# Autodesk Inventor assembly: benchtop-mesoSPIM-V2-1
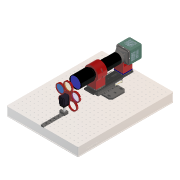
[picture p0: Inventor's stored thumbnail of the model, 180x180]
Saved by Autodesk Inventor 2021 (Build 250183000, 183)
## iProperties
Created: 2020-09-21
Part Number: benchtop-mesoSPIM-V2-1
Document SubType Name: Assembly
Designer: voigt
Author: voigt
## Documents named in this file (68)
- C:\Users\Public\GitHub-public\benchtop-hardware\Benchtop\CAD-model-Inventor2021\mesoSPIM\benchtop-mesoSPIM_latest.iam
- C:\Users\Public\GitHub-public\benchtop-hardware\Benchtop\CAD-model-Inventor2021\library\Thorlabs\breadboards\PBG52522-Step.iam
- C:\Users\Public\GitHub-public\benchtop-hardware\Benchtop\CAD-model-Inventor2021\library\Thorlabs\accessoires\AV6_M.ipt
- C:\Users\Public\GitHub-public\benchtop-hardware\Benchtop\CAD-model-Inventor2021\library\Thorlabs\extrusions\XE25L375_M.ipt
- C:\Users\Public\GitHub-public\benchtop-hardware\Benchtop\CAD-model-Inventor2021\library\Thorlabs\extrusions\RM1S.ipt
- C:\Users\Public\GitHub-public\benchtop-hardware\Benchtop\CAD-model-Inventor2021\library\Thorlabs\extrusions\RM1G.ipt
- C:\Users\Public\GitHub-public\benchtop-hardware\Benchtop\CAD-model-Inventor2021\library\Thorlabs\extrusions\XE25L525_M.ipt
- C:\Users\Public\GitHub-public\benchtop-hardware\Benchtop\CAD-model-Inventor2021\library\Thorlabs\extrusions\XE25L350_M.ipt
- C:\Users\Public\GitHub-public\benchtop-hardware\Benchtop\CAD-model-Inventor2021\library\Thorlabs\accessoires\BBH1.ipt
- C:\Users\Public\GitHub-public\benchtop-hardware\Benchtop\CAD-model-Inventor2021\mesoSPIM\covers\Front_Cover_V1.ipt
- C:\Users\Public\GitHub-public\benchtop-hardware\Benchtop\CAD-model-Inventor2021\library\ASI\LS100_Vertical_Assembly.ipt
- C:\Users\Public\GitHub-public\benchtop-hardware\Benchtop\CAD-model-Inventor2021\library\ASI\LS-50HE ASSEMBLY (Centered Travel).ipt
- C:\Users\Public\GitHub-public\benchtop-hardware\Benchtop\CAD-model-Inventor2021\library\ASI\VTS-2112 DOVE RACK ASSEMBLY - (#DV6010 and #DV6020)_DV6010 ASSEMBLY with CDZ-SLIDE C.iam
- C:\Users\Public\GitHub-public\benchtop-hardware\Benchtop\CAD-model-Inventor2021\library\ASI\LS-50 LE ASSEMBLY_HOME.iam
- C:\Users\Public\GitHub-public\benchtop-hardware\Benchtop\CAD-model-Inventor2021\library\ASI\C60-3060-CMR-1011 - C-MOUNT TO LS50 SLIDE ADAPTER.ipt
- C:\Users\Public\GitHub-public\benchtop-hardware\Benchtop\CAD-model-Inventor2021\library\ASI\C60-3060-CMR - 3060 C-MOUNT ROTATING ASSEMBLY_C60-3060-CMR-Mo-ER20.iam
- C:\Users\Public\GitHub-public\benchtop-hardware\Benchtop\CAD-model-Inventor2021\library\ASI\LS-5012 - LS-BREADBOARD ADAPTER PLATE.ipt
- C:\Users\Public\GitHub-public\benchtop-hardware\Benchtop\CAD-model-Inventor2021\library\Thorlabs\rails\XT66SD.ipt
- C:\Users\Public\GitHub-public\benchtop-hardware\Benchtop\CAD-model-Inventor2021\library\Photometrics\Iris15_Volume_Correct.ipt
- C:\Users\Public\GitHub-public\benchtop-hardware\Benchtop\CAD-model-Inventor2021\library\Thorlabs\rails\XT66P2_M_single.ipt
- C:\Users\Public\GitHub-public\benchtop-hardware\Benchtop\CAD-model-Inventor2021\mesoSPIM\covers\Side_Cover_V1.ipt
- C:\Users\Public\GitHub-public\benchtop-hardware\Benchtop\CAD-model-Inventor2021\mesoSPIM\covers\Top_Cover_V1.ipt
- C:\Users\Public\GitHub-public\benchtop-hardware\Benchtop\CAD-model-Inventor2021\library\Thorlabs\extrusions\XE25H.ipt
- C:\Users\Public\GitHub-public\benchtop-hardware\Benchtop\CAD-model-Inventor2021\library\Thorlabs\30mm_cage_system\cage_plates\CP33_M.ipt
- C:\Users\Public\GitHub-public\benchtop-hardware\Benchtop\CAD-model-Inventor2021\library\Thorlabs\30mm_cage_system\cage_rods\ER8_CageRod.ipt
- C:\Users\Public\GitHub-public\benchtop-hardware\Benchtop\CAD-model-Inventor2021\library\Thorlabs\optics\AC254-060-A-ML.ipt
- C:\Users\Public\GitHub-public\benchtop-hardware\Benchtop\CAD-model-Inventor2021\library\Thorlabs\accessoires\SM1FCA-APC-Fiberadapter.ipt
- C:\Users\Public\GitHub-public\benchtop-hardware\Benchtop\CAD-model-Inventor2021\library\Thorlabs\posts\post_mounts\PH40_M.ipt
- C:\Users\Public\GitHub-public\benchtop-hardware\Benchtop\CAD-model-Inventor2021\library\Thorlabs\posts\12_7_mm_posts\TR40M.ipt
- C:\Users\Public\GitHub-public\benchtop-hardware\Benchtop\CAD-model-Inventor2021\library\Thorlabs\30mm_cage_system\optics_mounts\KCB1E_M.ipt
- C:\Users\Public\GitHub-public\benchtop-hardware\Benchtop\CAD-model-Inventor2021\library\Thorlabs\optics\BBE1-E02-Step.ipt
- C:\Users\Public\GitHub-public\benchtop-hardware\Benchtop\CAD-model-Inventor2021\library\Thorlabs\optics\AC254-100-A-ML.ipt
- C:\Users\Public\GitHub-public\benchtop-hardware\Benchtop\CAD-model-Inventor2021\library\Optotune\EL-16-40\EL-16-40-TC-C (133-193-03-R0-01).iam
- C:\Users\Public\GitHub-public\benchtop-hardware\Benchtop\CAD-model-Inventor2021\library\Thorlabs\30mm_cage_system\SM1_tubes\SM1L10.ipt
- C:\Users\Public\GitHub-public\benchtop-hardware\Benchtop\CAD-model-Inventor2021\library\Thorlabs\accessoires\SM1A9.ipt
- C:\Users\Public\GitHub-public\benchtop-hardware\Benchtop\CAD-model-Inventor2021\library\Thorlabs\accessoires\SM1T2.ipt
- C:\Users\Public\GitHub-public\benchtop-hardware\Benchtop\CAD-model-Inventor2021\library\Thorlabs\accessoires\SM1NT.ipt
- C:\Users\Public\GitHub-public\benchtop-hardware\Benchtop\CAD-model-Inventor2021\library\Thorlabs\stages\XRN-B1_M-Micrometer-Baseplate.ipt
- C:\Users\Public\GitHub-public\benchtop-hardware\Benchtop\CAD-model-Inventor2021\library\Thorlabs\posts\post_mounts\PH75_M-Step.ipt
- C:\Users\Public\GitHub-public\benchtop-hardware\Benchtop\CAD-model-Inventor2021\library\Thorlabs\stages\XLN25P_M.ipt
- C:\Users\Public\GitHub-public\benchtop-hardware\Benchtop\CAD-model-Inventor2021\library\Thorlabs\stages\XRN25P_M.ipt
- C:\Users\Public\GitHub-public\benchtop-hardware\Benchtop\CAD-model-Inventor2021\library\Thorlabs\posts\12_7_mm_posts\TR75M.ipt
- C:\Users\Public\GitHub-public\benchtop-hardware\Benchtop\CAD-model-Inventor2021\mesoSPIM\excitation_path\components\60mm-blank-cageplate-LCP03M-Nikon-MOD.ipt
- C:\Users\Public\GitHub-public\benchtop-hardware\Benchtop\CAD-model-Inventor2021\library\Thorlabs\other\F-Mount-AdapterSM2NFM-Step.ipt
- C:\Users\Public\GitHub-public\benchtop-hardware\Benchtop\CAD-model-Inventor2021\library\Nikon\50mm_1_4G_body_disassembled.ipt
- C:\Users\Public\GitHub-public\benchtop-hardware\Benchtop\CAD-model-Inventor2021\library\Thorlabs\30mm_cage_system\cage_rods\ER4_CageRod.ipt
- C:\Users\Public\GitHub-public\benchtop-hardware\Benchtop\CAD-model-Inventor2021\mesoSPIM\sample_handling\Cuvette-Sampleholder\Cuvette-Sampleholder-with-base.iam
- C:\Users\nvladi\Documents\Inventor\mesoSPIM_design_benchtop_V2\library\Thorlabs\30mm_cage_system\cage_rods\ER_CageRod.ipt
- C:\Users\Public\GitHub-public\benchtop-hardware\Benchtop\CAD-model-Inventor2021\library\Mouse_Brain\mousebrain2.ipt
- C:\Users\Public\GitHub-public\benchtop-hardware\Benchtop\CAD-model-Inventor2021\mesoSPIM\immersion_cuvette_mounts\ImmersionCuvetteAssembly.iam
- C:\Users\Public\GitHub-public\benchtop-hardware\Benchtop\CAD-model-Inventor2021\mesoSPIM\sample_handling\IDISCO-Sampleholder\Clamp-assembly.iam
- C:\Users\Public\GitHub-public\benchtop-hardware\Benchtop\CAD-model-Inventor2021\library\Thorlabs\accessoires\SM1A10.ipt
- C:\Users\Public\GitHub-public\benchtop-hardware\Benchtop\CAD-model-Inventor2021\library\Thorlabs\accessoires\SM1M20.ipt
- C:\Users\Public\GitHub-public\benchtop-hardware\Benchtop\CAD-model-Inventor2021\library\Thorlabs\optics\AC254-060-A-ML_CPY.ipt
- C:\Users\Public\GitHub-public\benchtop-hardware\Benchtop\CAD-model-Inventor2021\library\Thorlabs\accessoires\SM1FCA-APC-Fiberadapter_CPY.ipt
- C:\Users\Public\GitHub-public\benchtop-hardware\Benchtop\CAD-model-Inventor2021\mesoSPIM\detection_path\filter-wheel\FilterWheel-Dynamixel(MX28).iam
- C:\Users\Public\GitHub-public\benchtop-hardware\Benchtop\CAD-model-Inventor2021\library\Thorlabs\rails\RLA150_M.ipt
- C:\Users\Public\GitHub-public\benchtop-hardware\Benchtop\custom-parts\excitation-mirror-bracket\mirror-bracket.ipt
- C:\Users\Public\GitHub-public\benchtop-hardware\Benchtop\CAD-model-Inventor2021\mesoSPIM\excitation_path\15mm-galvo(Thorlabs-QS15)-assembly\15mm-QS15-galvo-assembly.iam
- C:\Users\Public\GitHub-public\benchtop-hardware\Benchtop\CAD-model-Inventor2021\library\ASI\ASI_mesoSPIM_Bridge-wide.ipt
- C:\Users\Public\GitHub-public\benchtop-hardware\Benchtop\CAD-model-Inventor2021\mesoSPIM\detection_path\Mitutoyo\Mitutoyo-BD-Plan-Apo-system.iam
- C:\Users\Public\GitHub-public\benchtop-hardware\Benchtop\custom-parts\detection-objective-mounts\Iris15-XT66P2M.ipt
- C:\Users\Public\GitHub-public\benchtop-hardware\Benchtop\CAD-model-Inventor2021\library\Thorlabs\accessoires\AB90H.ipt
- C:\Users\Public\GitHub-public\benchtop-hardware\Benchtop\custom-parts\detection-objective-mounts\ThorlabsSM2L30-XT66P2M.ipt
- C:\Users\Public\GitHub-public\benchtop-hardware\Benchtop\custom-parts\detection-accessories\Mitutoyo-MT1(tube-lens)-SM2-adapter\AdapterMT1-SM2tube.ipt
- C:\Users\Public\GitHub-public\benchtop-hardware\Benchtop\CAD-model-Inventor2021\library\Thorlabs\kinematic_bases\KB25_M-Step.ipt
- C:\Users\Public\GitHub-public\benchtop-hardware\Benchtop\CAD-model-Inventor2021\library\Lensation\Lensagon-T25M-12-155I.ipt
- C:\Users\Public\GitHub-public\benchtop-hardware\Benchtop\CAD-model-Inventor2021\mesoSPIM\detection_path\filter-wheel\Filter.ipt
## Components (146 placed, 66 different names)
1. Filter:1 — Flush:83
2. Filter:2 — Insert:27
3. Filter:3 — Insert:26
4. AV6_M:4 — Mate:6, Mate:7
5. AV6_M:3 — Mate:8, Mate:9
6. AV6_M:2 — Mate:12, Mate:13
7. AV6_M:1 — Mate:10, Mate:11
8. PBG52522-Step:1 [sub-assembly] — Flush:1, Flush:2, Mate:5, Mate:6, Mate:7, Mate:8, Mate:9, Mate:10, Mate:11, Mate:12, Mate:13, Mate:14, Mate:15, Angle:1, Mate:16, Mate:17, Angle:2, Mate:18, Mate:19, Angle:3, Mate:20, Mate:21, Angle:4, Mate:32, Mate:48, Mate:49, Angle:5, Angle:6, Mate:72, Flush:45, Mate:139, Mate:140, Angle:18, Mate:141, Mate:142, Angle:19, Flush:49, Angle:20, Mate:191, Mate:192, Angle:23, Angle:24, Mate:196, Mate:197, Mate:198, Angle:25, Mate:199, Mate:200, Angle:26, Mate:238, Mate:239, Angle:28, Angle:30, Mate:243, Angle:44, Mate:385, Angle:47, Insert:19, Angle:48, Angle:49, Angle:50, Flush:74, Flush:75, Mate:392, Mate:395, Mate:397, Mate:398
9. TR40M:5 — Mate:367, VerticalPos, Insert:9
10. LS100_Vertical_Assembly:1 — Mate:48, Angle:5, Mate:52, Flush:74, Mate:391, Mate:393, Mate:394, Flush:78
11. LS100_Vertical_Assembly:2 — Mate:49, Angle:6, Flush:75, Mate:396, Flush:79, Mate:399, Flush:80
12. ASI_mesoSPIM_Bridge-wide:1 — Mate:52, Mate:55, Flush:36
13. LS-50HE ASSEMBLY (Centered Travel):1 — Mate:55, Flush:36, Mate:56, Mate:57, Angle:7, Mate:58, Mate:59, Angle:8
14. AB90H:1 — Mate:394, Mate:395, Flush:78
15. AB90H:2 — Mate:391, Mate:392, Mate:393
16. AB90H:3 — Mate:396, Flush:79, Mate:397
17. AB90H:4 — Mate:398, Mate:399, Flush:80
18. VTS-2112 DOVE RACK ASSEMBLY - (#DV6010 and #DV6020)_DV6010 ASSEMBLY with CDZ-SLIDE C:1 [sub-assembly] — Mate:57, Angle:7, Mate:58, Mate:59, Mate:60, Mate:61, Mate:62
19. LS-50 LE ASSEMBLY_HOME:1 [sub-assembly] — Mate:60, Mate:61, Mate:62, Angle:8, Mate:63, Mate:64, Mate:65
20. C60-3060-CMR-1011 - C-MOUNT TO LS50 SLIDE ADAPTER:1 — Mate:63, Mate:64, Mate:65, Mate:66, Mate:67
21. C60-3060-CMR - 3060 C-MOUNT ROTATING ASSEMBLY_C60-3060-CMR-Mo-ER20:1 [sub-assembly] — Mate:66, Mate:67, Mate:367, VerticalPos
22. AdapterMT1-SM2tube:1
23. ThorlabsSM2L30-XT66P2M:1 — Mate:400, Flush:81, Flush:82
24. Lensagon-T25M-12-155I:1 — Insert:25
25. Mitutoyo-BD-Plan-Apo-system:1 [sub-assembly] — Insert:24
26. Iris15-XT66P2M:1 — Mate:390, Flush:76, Flush:77
27. Iris15_Volume_Correct:1 — Angle:11, Insert:24, Insert:25
28. XT66P2_M_single:1 — Mate:82, Mate:83, Mate:390, Flush:76, Flush:77
29. XT66P2_M_single:2 — Mate:84, Mate:85, Mate:400, Flush:81, Flush:82
30. 15mm-QS15-galvo-assembly:1 [sub-assembly] — Insert:21
31. mirror-bracket:1 — Mate:389, Angle:50
32. SM1M20:1 — Insert:15, Insert:17
33. SM1A10:1 — Insert:12, Insert:14
34. SM1FCA-APC-Fiberadapter:1 — Insert:17
35. AC254-060-A-ML:1 — Insert:14, Insert:15
36. 60mm-blank-cageplate-LCP03M-Nikon-MOD:1 — Mate:344, Mate:345, Mate:347, Flush:66, Mate:350, Flush:67, Insert:1
37. F-Mount-AdapterSM2NFM-Step:1 — Mate:344, Mate:345, Mate:346
38. 50mm_1_4G_body_disassembled:1 — Mate:346, Mate:347
39. TR75M:2 — Mate:272
40. KCB1E_M:4 — Mate:254, Mate:255, Mate:258, Mate:259, Mate:389
41. BBE1-E02-Step:5 — Mate:258, Mate:259
42. XRN25P_M:2
43. PH75_M-Step:2 — Mate:192, Angle:23, Mate:272
44. XRN-B1_M-Micrometer-Baseplate:1 — Mate:191, Angle:24, Mate:196
45. EL-16-40-TC-C (133-193-03-R0-01):1 [sub-assembly] — Mate:175, Mate:178, Mate:179, Insert:12
46. SM1L10:2 — Mate:177, Mate:181, Mate:182, Mate:183
47. SM1A9:1 — Mate:178, Mate:179, Mate:180
48. SM1T2:1 — Mate:180, Mate:181
49. SM1NT:1 — Mate:182, Mate:183
50. PH40_M:1 — Mate:139, Mate:140, Angle:18, Mate:148
51. PH40_M:2 — Mate:141, Mate:142, Angle:19, Mate:150
52. CP33_M:5 — Mate:147, Mate:148, Mate:153, Mate:154, Mate:155, Mate:156, Flush:53, Mate:159, Mate:160, Angle:51
53. CP33_M:6 — Mate:149, Mate:150, Mate:161, Mate:162
54. CP33_M:13 — Insert:22, Insert:23, Angle:51
55. CP33_M:7 — Mate:151, Mate:157, Flush:54, Mate:169
56. ER8_CageRod:4 — Mate:156, Flush:51
57. ER8_CageRod:5 — Mate:155, Flush:50, Flush:51, Flush:52, Mate:157, Insert:23
58. ER8_CageRod:6 — Mate:154, Flush:52
59. ER8_CageRod:7 — Mate:153, Flush:50, Flush:53, Flush:54, Mate:164, Mate:165
60. TR40M:1 — Mate:159, Mate:160
61. TR40M:2 — Mate:161, Mate:162
62. KCB1E_M:1 — Mate:163, Mate:164, Mate:165, Mate:167, Mate:175, Mate:177
63. BBE1-E02-Step:1 — Mate:166, Mate:167, Angle:20
64. AC254-100-A-ML:1 — Mate:168, Mate:169
65. AC254-100-A-ML:2 — Insert:22
66. ER4_CageRod:12 — Flush:66
67. ER4_CageRod:19 — Insert:1
68. ER4_CageRod:20
69. ER4_CageRod:13 — Mate:350, Flush:67, Insert:21
70. 15mm-QS15-galvo-assembly:2 [sub-assembly] — Insert:20
71. mirror-bracket:2 — Mate:388, Angle:49
72. SM1FCA-APC-Fiberadapter_CPY:1 — Insert:18
73. AC254-060-A-ML_CPY:1 — Insert:16
74. SM1M20:2 — Insert:16, Insert:18
75. SM1A10:2 — Insert:13
76. 60mm-blank-cageplate-LCP03M-Nikon-MOD:2 — Mate:358, Mate:359, Mate:361, Mate:365, Flush:70, Flush:71, Mate:366
77. F-Mount-AdapterSM2NFM-Step:2 — Mate:358, Mate:359, Mate:360
78. 50mm_1_4G_body_disassembled:2 — Mate:360, Mate:361
79. ER4_CageRod:14 — Mate:365, Flush:70
80. ER4_CageRod:16 — Flush:71, Mate:366, Insert:20
81. TR75M:4 — Mate:278
82. KCB1E_M:5 — Mate:256, Mate:261, Mate:388
83. BBE1-E02-Step:4 — Mate:261
84. XLN25P_M:1 — Mate:403
85. PH40_M:3 — Mate:197, Mate:198, Angle:25, Mate:205
86. PH40_M:4 — Mate:199, Mate:200, Angle:26, Mate:206
87. CP33_M:9 — Mate:201, Mate:205, Mate:207, Mate:208, Mate:211, Mate:212, Mate:213, Mate:214
88. CP33_M:10 — Mate:202, Mate:206, Mate:209, Mate:210, Flush:58
89. TR40M:3 — Mate:207, Mate:208
90. TR40M:4 — Mate:209, Mate:210
91. ER8_CageRod:8 — Mate:211, Flush:57, Flush:59
92. ER8_CageRod:9 — Mate:213, Flush:56, Flush:58, Mate:216, Mate:217, Mate:222
93. ER8_CageRod:10 — Mate:214, Flush:55, Flush:56, Flush:57
94. ER8_CageRod:11 — Mate:212, Flush:55
95. ER4_CageRod:21
96. ER4_CageRod:22
97. KCB1E_M:3 — Mate:215, Mate:216, Mate:217, Mate:219, Angle:27, Mate:227, Mate:228, Mate:229, Mate:231
98. BBE1-E02-Step:3 — Mate:218, Mate:219, Angle:27
99. CP33_M:11 — Mate:220, Flush:59, Mate:224
100. CP33_M:12 — Mate:221, Mate:222, Mate:226
101. AC254-100-A-ML:3 — Mate:223, Mate:224
102. AC254-100-A-ML:4 — Mate:225, Mate:226, Mate:227
103. SM1L10:3 — Mate:228, Mate:229, Mate:230, Mate:236, Mate:237
104. EL-16-40-TC-C (133-193-03-R0-01):2 [sub-assembly] — Mate:230, Mate:231, Mate:232, Mate:233, Insert:13
105. SM1A9:3 — Mate:232, Mate:233, Mate:234, Mate:235
106. SM1T2:2 — Mate:234, Mate:235
107. SM1NT:2 — Mate:236, Mate:237
108. XRN-B1_M-Micrometer-Baseplate:2 — Mate:238, Angle:30, Mate:243, Mate:403
109. PH75_M-Step:3 — Mate:239, Angle:28, Mate:278
110. mousebrain2:1
111. ImmersionCuvetteAssembly:1 [sub-assembly] — Mate:385
112. Clamp-assembly:1 [sub-assembly] — Insert:9, Angle:47
113. KB25_M-Step:1
114. Cuvette-Sampleholder-with-base:1 [sub-assembly] — Angle:44
115. RLA150_M:1 — Insert:19, Angle:48, Mate:386, Mate:387
116. FilterWheel-Dynamixel(MX28):1 [sub-assembly] — Mate:386, Mate:387, Flush:83, Insert:26, Insert:27
117. XE25H:1 — Mate:103, Angle:14, Mate:104, Flush:43
118. XE25H:2 — Mate:105, Mate:106, Flush:44
119. XE25L525_M:1 — Mate:29, Flush:17, Flush:18, Mate:101, Flush:40, Flush:42
120. XE25L525_M:2 — Mate:28, Flush:15, Flush:16, Mate:100, Flush:38
121. XE25L375_M:5 — Mate:27, Flush:13, Flush:14, Flush:19, Mate:30, Flush:20, Mate:103, Flush:43, Mate:105, Flush:44
122. XE25L375_M:6 — Mate:26, Flush:11, Flush:12, Flush:41
123. RM1G:1 — Mate:22, Flush:3, Flush:4, Mate:28, Flush:15, Flush:16
124. RM1G:2 — Mate:24, Flush:7, Flush:8, Mate:26, Flush:11, Flush:12, Mate:29, Flush:17, Flush:18
125. RM1G:3 — Mate:25, Flush:9, Flush:10, Mate:27, Flush:13, Flush:14, Mate:104
126. RM1G:4 — Mate:23, Flush:5, Flush:6, Mate:102, Mate:106
127. XE25L375_M:1 — Mate:14, Mate:15, Angle:1, Mate:22, Flush:3, Flush:4, Flush:37
128. XE25L375_M:2 — Mate:16, Mate:17, Angle:2, Mate:24, Flush:7, Flush:8, Flush:39
129. XE25L375_M:3 — Mate:18, Mate:19, Angle:3, Mate:25, Flush:9, Flush:10
130. XE25L375_M:4 — Mate:20, Mate:21, Angle:4, Mate:23, Flush:5, Flush:6, Flush:21, Mate:31
131. Front_Cover_V1:1 — Mate:41, Mate:42, Mate:43
132. BBH1:1 — Mate:39, Flush:35, Mate:40
133. RM1S:1 — Mate:33, Flush:22, Flush:23
134. RM1S:2 — Mate:34, Flush:24, Flush:25, Flush:33, Flush:34, Mate:38
135. RM1S:3 — Flush:28, Mate:36, Flush:29, Flush:30, Mate:37, Flush:31, Flush:32
136. RM1S:4 — Mate:35, Flush:26, Flush:27
137. XE25L375_M:7 — Flush:19, Mate:30, Flush:20, Mate:34, Flush:24, Flush:25, Flush:28, Mate:36, Flush:29, Flush:30, Mate:43, Angle:14
138. XE25L375_M:8 — Flush:21, Mate:31, Mate:32, Mate:33, Flush:22, Flush:23, Mate:35, Flush:26, Flush:27, Mate:39, Flush:35
139. XE25L350_M:1 — Mate:37, Flush:31, Flush:32, Mate:41, Mate:42
140. XE25L350_M:2 — Flush:33, Flush:34, Mate:38
141. Side_Cover_V1:1 — Mate:100, Flush:37, Flush:38
142. Side_Cover_V1:2 — Mate:101, Flush:39, Flush:40
143. Top_Cover_V1:1 — Mate:102, Flush:41, Flush:42
144. LS-5012 - LS-BREADBOARD ADAPTER PLATE:1 — Mate:70, Angle:9, Mate:72, Mate:77
145. LS-50 LE ASSEMBLY_HOME:2 [sub-assembly] — Mate:70, Angle:9, Mate:73, Mate:74, Angle:10, Mate:77
146. XT66SD:1 — Mate:73, Mate:74, Angle:10, Mate:75, Mate:76, Angle:11, Mate:82, Mate:83, Mate:84, Mate:85
## Relationships (325: Mate 206, Flush 72, Angle 29, Insert 18)
- Flush:1 (135 mm): PBG52522-Step:1
- Flush:2 (225 mm): PBG52522-Step:1
- Mate:5 (-100 mm): PBG52522-Step:1
- Mate:6: AV6_M:4 ↔ PBG52522-Step:1
- Mate:7: AV6_M:4 ↔ PBG52522-Step:1
- Mate:8: AV6_M:3 ↔ PBG52522-Step:1
- Mate:9: AV6_M:3 ↔ PBG52522-Step:1
- Mate:10: AV6_M:1 ↔ PBG52522-Step:1
- Mate:11: AV6_M:1 ↔ PBG52522-Step:1
- Mate:12: AV6_M:2 ↔ PBG52522-Step:1
- Mate:13: AV6_M:2 ↔ PBG52522-Step:1
- Mate:14: PBG52522-Step:1 ↔ XE25L375_M:1
- Mate:15: PBG52522-Step:1 ↔ XE25L375_M:1
- Angle:1 (0 deg): PBG52522-Step:1 ↔ XE25L375_M:1
- Mate:16: PBG52522-Step:1 ↔ XE25L375_M:2
- Mate:17: PBG52522-Step:1 ↔ XE25L375_M:2
- Angle:2 (0 deg): PBG52522-Step:1 ↔ XE25L375_M:2
- Mate:18: PBG52522-Step:1 ↔ XE25L375_M:3
- Mate:19: PBG52522-Step:1 ↔ XE25L375_M:3
- Angle:3 (0 deg): PBG52522-Step:1 ↔ XE25L375_M:3
- Mate:20: PBG52522-Step:1 ↔ XE25L375_M:4
- Mate:21: PBG52522-Step:1 ↔ XE25L375_M:4
- Angle:4 (0 deg): PBG52522-Step:1 ↔ XE25L375_M:4
- Mate:22: RM1G:1 ↔ XE25L375_M:1
- Flush:3: RM1G:1 ↔ XE25L375_M:1
- Flush:4: RM1G:1 ↔ XE25L375_M:1
- Mate:23: RM1G:4 ↔ XE25L375_M:4
- Flush:5: RM1G:4 ↔ XE25L375_M:4
- Flush:6: RM1G:4 ↔ XE25L375_M:4
- Mate:24: RM1G:2 ↔ XE25L375_M:2
- Flush:7: RM1G:2 ↔ XE25L375_M:2
- Flush:8: RM1G:2 ↔ XE25L375_M:2
- Mate:25: RM1G:3 ↔ XE25L375_M:3
- Flush:9: RM1G:3 ↔ XE25L375_M:3
- Flush:10: RM1G:3 ↔ XE25L375_M:3
- Mate:26: XE25L375_M:6 ↔ RM1G:2
- Flush:11: XE25L375_M:6 ↔ RM1G:2
- Flush:12: XE25L375_M:6 ↔ RM1G:2
- Mate:27: XE25L375_M:5 ↔ RM1G:3
- Flush:13: XE25L375_M:5 ↔ RM1G:3
- Flush:14: XE25L375_M:5 ↔ RM1G:3
- Mate:28: XE25L525_M:2 ↔ RM1G:1
- Flush:15: XE25L525_M:2 ↔ RM1G:1
- Flush:16: XE25L525_M:2 ↔ RM1G:1
- Mate:29: XE25L525_M:1 ↔ RM1G:2
- Flush:17: XE25L525_M:1 ↔ RM1G:2
- Flush:18: XE25L525_M:1 ↔ RM1G:2
- Flush:19: XE25L375_M:5 ↔ XE25L375_M:7
- Mate:30: XE25L375_M:5 ↔ XE25L375_M:7
- Flush:20: XE25L375_M:5 ↔ XE25L375_M:7
- Flush:21 (-25 mm): XE25L375_M:4 ↔ XE25L375_M:8
- Mate:31: XE25L375_M:4 ↔ XE25L375_M:8
- Mate:32: PBG52522-Step:1 ↔ XE25L375_M:8
- Mate:33: RM1S:1 ↔ XE25L375_M:8
- Flush:22: RM1S:1 ↔ XE25L375_M:8
- Flush:23: RM1S:1 ↔ XE25L375_M:8
- Mate:34: RM1S:2 ↔ XE25L375_M:7
- Flush:24: RM1S:2 ↔ XE25L375_M:7
- Flush:25: RM1S:2 ↔ XE25L375_M:7
- Mate:35: RM1S:4 ↔ XE25L375_M:8
- Flush:26: RM1S:4 ↔ XE25L375_M:8
- Flush:27: RM1S:4 ↔ XE25L375_M:8
- Flush:28: RM1S:3 ↔ XE25L375_M:7
- Mate:36: RM1S:3 ↔ XE25L375_M:7
- Flush:29: RM1S:3 ↔ XE25L375_M:7
- Flush:30: RM1S:3 ↔ XE25L375_M:7
- Mate:37: RM1S:3 ↔ XE25L350_M:1
- Flush:31: RM1S:3 ↔ XE25L350_M:1
- Flush:32: RM1S:3 ↔ XE25L350_M:1
- Flush:33: RM1S:2 ↔ XE25L350_M:2
- Flush:34: RM1S:2 ↔ XE25L350_M:2
- Mate:38: RM1S:2 ↔ XE25L350_M:2
- Mate:39: BBH1:1 ↔ XE25L375_M:8
- Flush:35: BBH1:1 ↔ XE25L375_M:8
- Mate:40 (62.5 mm): BBH1:1
- Mate:41: Front_Cover_V1:1 ↔ XE25L350_M:1
- Mate:42 (-6 mm): Front_Cover_V1:1 ↔ XE25L350_M:1
- Mate:43 (-2 mm): Front_Cover_V1:1 ↔ XE25L375_M:7
- Mate:44
- Mate:45
- Mate:48: PBG52522-Step:1 ↔ LS100_Vertical_Assembly:1
- Mate:49: PBG52522-Step:1 ↔ LS100_Vertical_Assembly:2
- Angle:5 (0 deg): PBG52522-Step:1 ↔ LS100_Vertical_Assembly:1
- Angle:6 (0 deg): PBG52522-Step:1 ↔ LS100_Vertical_Assembly:2
- Mate:52: LS100_Vertical_Assembly:1 ↔ ASI_mesoSPIM_Bridge-wide:1
- Mate:55: ASI_mesoSPIM_Bridge-wide:1 ↔ LS-50HE ASSEMBLY (Centered Travel):1
- Flush:36: ASI_mesoSPIM_Bridge-wide:1 ↔ LS-50HE ASSEMBLY (Centered Travel):1
- Mate:56 (12.5 mm): LS-50HE ASSEMBLY (Centered Travel):1
- Mate:57: LS-50HE ASSEMBLY (Centered Travel):1 ↔ VTS-2112 DOVE RACK ASSEMBLY - (#DV6010 and #DV6020)_DV6010 ASSEMBLY with CDZ-SLIDE C:1
- Angle:7 (0 deg): LS-50HE ASSEMBLY (Centered Travel):1 ↔ VTS-2112 DOVE RACK ASSEMBLY - (#DV6010 and #DV6020)_DV6010 ASSEMBLY with CDZ-SLIDE C:1
- Mate:58: LS-50HE ASSEMBLY (Centered Travel):1 ↔ VTS-2112 DOVE RACK ASSEMBLY - (#DV6010 and #DV6020)_DV6010 ASSEMBLY with CDZ-SLIDE C:1
- Mate:59: LS-50HE ASSEMBLY (Centered Travel):1 ↔ VTS-2112 DOVE RACK ASSEMBLY - (#DV6010 and #DV6020)_DV6010 ASSEMBLY with CDZ-SLIDE C:1
- Mate:60: VTS-2112 DOVE RACK ASSEMBLY - (#DV6010 and #DV6020)_DV6010 ASSEMBLY with CDZ-SLIDE C:1 ↔ LS-50 LE ASSEMBLY_HOME:1
- Mate:61: VTS-2112 DOVE RACK ASSEMBLY - (#DV6010 and #DV6020)_DV6010 ASSEMBLY with CDZ-SLIDE C:1 ↔ LS-50 LE ASSEMBLY_HOME:1
- Mate:62: VTS-2112 DOVE RACK ASSEMBLY - (#DV6010 and #DV6020)_DV6010 ASSEMBLY with CDZ-SLIDE C:1 ↔ LS-50 LE ASSEMBLY_HOME:1
- Angle:8 (0 deg): LS-50HE ASSEMBLY (Centered Travel):1 ↔ LS-50 LE ASSEMBLY_HOME:1
- Mate:63: LS-50 LE ASSEMBLY_HOME:1 ↔ C60-3060-CMR-1011 - C-MOUNT TO LS50 SLIDE ADAPTER:1
- Mate:64: LS-50 LE ASSEMBLY_HOME:1 ↔ C60-3060-CMR-1011 - C-MOUNT TO LS50 SLIDE ADAPTER:1
- Mate:65: LS-50 LE ASSEMBLY_HOME:1 ↔ C60-3060-CMR-1011 - C-MOUNT TO LS50 SLIDE ADAPTER:1
- Mate:66: C60-3060-CMR-1011 - C-MOUNT TO LS50 SLIDE ADAPTER:1 ↔ C60-3060-CMR - 3060 C-MOUNT ROTATING ASSEMBLY_C60-3060-CMR-Mo-ER20:1
- Mate:67: C60-3060-CMR-1011 - C-MOUNT TO LS50 SLIDE ADAPTER:1 ↔ C60-3060-CMR - 3060 C-MOUNT ROTATING ASSEMBLY_C60-3060-CMR-Mo-ER20:1
- Mate:70: LS-5012 - LS-BREADBOARD ADAPTER PLATE:1 ↔ LS-50 LE ASSEMBLY_HOME:2
- Angle:9 (0 deg): LS-5012 - LS-BREADBOARD ADAPTER PLATE:1 ↔ LS-50 LE ASSEMBLY_HOME:2
- Mate:72: PBG52522-Step:1 ↔ LS-5012 - LS-BREADBOARD ADAPTER PLATE:1
- Mate:73: LS-50 LE ASSEMBLY_HOME:2 ↔ XT66SD:1
- Mate:74: LS-50 LE ASSEMBLY_HOME:2 ↔ XT66SD:1
- Angle:10 (0 deg): LS-50 LE ASSEMBLY_HOME:2 ↔ XT66SD:1
- Mate:75: XT66SD:1
- Mate:76: XT66SD:1
- Mate:77: LS-5012 - LS-BREADBOARD ADAPTER PLATE:1 ↔ LS-50 LE ASSEMBLY_HOME:2
- Angle:11 (0 deg): Iris15_Volume_Correct:1 ↔ XT66SD:1
- Mate:82: XT66P2_M_single:1 ↔ XT66SD:1
- Mate:83: XT66P2_M_single:1 ↔ XT66SD:1
- Mate:84: XT66P2_M_single:2 ↔ XT66SD:1
- Mate:85: XT66P2_M_single:2 ↔ XT66SD:1
- Mate:100: XE25L525_M:2 ↔ Side_Cover_V1:1
- Flush:37: XE25L375_M:1 ↔ Side_Cover_V1:1
- Flush:38: XE25L525_M:2 ↔ Side_Cover_V1:1
- Mate:101: XE25L525_M:1 ↔ Side_Cover_V1:2
- Flush:39: XE25L375_M:2 ↔ Side_Cover_V1:2
- Flush:40: XE25L525_M:1 ↔ Side_Cover_V1:2
- Mate:102: RM1G:4 ↔ Top_Cover_V1:1
- Flush:41: XE25L375_M:6 ↔ Top_Cover_V1:1
- Flush:42: XE25L525_M:1 ↔ Top_Cover_V1:1
- Mate:103: XE25H:1 ↔ XE25L375_M:5
- Angle:14 (0 deg): XE25H:1 ↔ XE25L375_M:7
- Mate:104: XE25H:1 ↔ RM1G:3
- Flush:43 (5.75 mm): XE25H:1 ↔ XE25L375_M:5
- Mate:105: XE25H:2 ↔ XE25L375_M:5
- Mate:106: XE25H:2 ↔ RM1G:4
- Flush:44 (5.75 mm): XE25H:2 ↔ XE25L375_M:5
- Flush:45 (215 mm): PBG52522-Step:1
- Flush:46 (-100 mm)
- Flush:47 (100 mm)
- Mate:139: PBG52522-Step:1 ↔ PH40_M:1
- Mate:140: PBG52522-Step:1 ↔ PH40_M:1
- Angle:18 (0 deg): PBG52522-Step:1 ↔ PH40_M:1
- Mate:141: PBG52522-Step:1 ↔ PH40_M:2
- Mate:142: PBG52522-Step:1 ↔ PH40_M:2
- Angle:19 (0 deg): PBG52522-Step:1 ↔ PH40_M:2
- Flush:49 (70 mm): PBG52522-Step:1
- Mate:143
- Mate:144
- Mate:145
- Mate:146
- Mate:147: CP33_M:5
- Mate:148: PH40_M:1 ↔ CP33_M:5
- Mate:149: CP33_M:6
- Mate:150: PH40_M:2 ↔ CP33_M:6
- Mate:151: CP33_M:7
- Mate:153: CP33_M:5 ↔ ER8_CageRod:7
- Mate:154: CP33_M:5 ↔ ER8_CageRod:6
- Mate:155: CP33_M:5 ↔ ER8_CageRod:5
- Mate:156: CP33_M:5 ↔ ER8_CageRod:4
- Flush:50: ER8_CageRod:5 ↔ ER8_CageRod:7
- Flush:51: ER8_CageRod:4 ↔ ER8_CageRod:5
- Flush:52: ER8_CageRod:5 ↔ ER8_CageRod:6
- Flush:53 (-39 mm): CP33_M:5 ↔ ER8_CageRod:7
- Mate:157: CP33_M:7 ↔ ER8_CageRod:5
- Mate:159: CP33_M:5 ↔ TR40M:1
- Mate:160: CP33_M:5 ↔ TR40M:1
- Mate:161: CP33_M:6 ↔ TR40M:2
- Mate:162: CP33_M:6 ↔ TR40M:2
- Flush:54: CP33_M:7 ↔ ER8_CageRod:7
- Mate:163: KCB1E_M:1
- Mate:164: ER8_CageRod:7 ↔ KCB1E_M:1
- Mate:165: ER8_CageRod:7 ↔ KCB1E_M:1
- Mate:166: BBE1-E02-Step:1
- Mate:167: KCB1E_M:1 ↔ BBE1-E02-Step:1
- Angle:20 (-90 deg): PBG52522-Step:1 ↔ BBE1-E02-Step:1
- Mate:168: AC254-100-A-ML:1
- Mate:169: CP33_M:7 ↔ AC254-100-A-ML:1
- Mate:175 (35.6 mm): EL-16-40-TC-C (133-193-03-R0-01):1 ↔ KCB1E_M:1
- Mate:177: SM1L10:2 ↔ KCB1E_M:1
- Mate:178: EL-16-40-TC-C (133-193-03-R0-01):1 ↔ SM1A9:1
- Mate:179: EL-16-40-TC-C (133-193-03-R0-01):1 ↔ SM1A9:1
- Mate:180: SM1A9:1 ↔ SM1T2:1
- Mate:181: SM1L10:2 ↔ SM1T2:1
- Mate:182: SM1L10:2 ↔ SM1NT:1
- Mate:183: SM1L10:2 ↔ SM1NT:1
- Mate:191: PBG52522-Step:1 ↔ XRN-B1_M-Micrometer-Baseplate:1
- Mate:192: PBG52522-Step:1 ↔ PH75_M-Step:2
- Angle:23 (0 deg): PBG52522-Step:1 ↔ PH75_M-Step:2
- Angle:24 (0 deg): PBG52522-Step:1 ↔ XRN-B1_M-Micrometer-Baseplate:1
- Mate:196: PBG52522-Step:1 ↔ XRN-B1_M-Micrometer-Baseplate:1
- Mate:197: PBG52522-Step:1 ↔ PH40_M:3
- Mate:198: PBG52522-Step:1 ↔ PH40_M:3
- Angle:25 (0 deg): PBG52522-Step:1 ↔ PH40_M:3
- Mate:199: PBG52522-Step:1 ↔ PH40_M:4
- Mate:200: PBG52522-Step:1 ↔ PH40_M:4
- Angle:26 (0 deg): PBG52522-Step:1 ↔ PH40_M:4
- Mate:201: CP33_M:9
- Mate:202: CP33_M:10
- Mate:205: PH40_M:3 ↔ CP33_M:9
- Mate:206: PH40_M:4 ↔ CP33_M:10
- Mate:207: CP33_M:9 ↔ TR40M:3
- Mate:208: CP33_M:9 ↔ TR40M:3
- Mate:209: CP33_M:10 ↔ TR40M:4
- Mate:210: CP33_M:10 ↔ TR40M:4
- Mate:211: CP33_M:9 ↔ ER8_CageRod:8
- Mate:212: CP33_M:9 ↔ ER8_CageRod:11
- Mate:213: CP33_M:9 ↔ ER8_CageRod:9
- Mate:214: CP33_M:9 ↔ ER8_CageRod:10
- Flush:55: ER8_CageRod:10 ↔ ER8_CageRod:11
- Flush:56: ER8_CageRod:9 ↔ ER8_CageRod:10
- Flush:57: ER8_CageRod:8 ↔ ER8_CageRod:10
- Flush:58 (-39 mm): CP33_M:10 ↔ ER8_CageRod:9
- Mate:215: KCB1E_M:3
- Mate:216: ER8_CageRod:9 ↔ KCB1E_M:3
- Mate:217: ER8_CageRod:9 ↔ KCB1E_M:3
- Mate:218: BBE1-E02-Step:3
- Mate:219: KCB1E_M:3 ↔ BBE1-E02-Step:3
- Angle:27 (0 deg): KCB1E_M:3 ↔ BBE1-E02-Step:3
- Mate:220: CP33_M:11
- Mate:221: CP33_M:12
- Mate:222: ER8_CageRod:9 ↔ CP33_M:12
- Flush:59: ER8_CageRod:8 ↔ CP33_M:11
- Mate:223: AC254-100-A-ML:3
- Mate:224: CP33_M:11 ↔ AC254-100-A-ML:3
- Mate:225: AC254-100-A-ML:4
- Mate:226: CP33_M:12 ↔ AC254-100-A-ML:4
- Mate:227 (0.5 mm): KCB1E_M:3 ↔ AC254-100-A-ML:4
- Mate:228: KCB1E_M:3 ↔ SM1L10:3
- Mate:229: KCB1E_M:3 ↔ SM1L10:3
- Mate:230: SM1L10:3 ↔ EL-16-40-TC-C (133-193-03-R0-01):2
- Mate:231 (35.6 mm): KCB1E_M:3 ↔ EL-16-40-TC-C (133-193-03-R0-01):2
- Mate:232: EL-16-40-TC-C (133-193-03-R0-01):2 ↔ SM1A9:3
- Mate:233: EL-16-40-TC-C (133-193-03-R0-01):2 ↔ SM1A9:3
- Mate:234: SM1A9:3 ↔ SM1T2:2
- Mate:235: SM1A9:3 ↔ SM1T2:2
- Mate:236: SM1L10:3 ↔ SM1NT:2
- Mate:237: SM1L10:3 ↔ SM1NT:2
- Mate:238: PBG52522-Step:1 ↔ XRN-B1_M-Micrometer-Baseplate:2
- Mate:239: PBG52522-Step:1 ↔ PH75_M-Step:3
- Angle:28 (0 deg): PBG52522-Step:1 ↔ PH75_M-Step:3
- Angle:30 (0 deg): PBG52522-Step:1 ↔ XRN-B1_M-Micrometer-Baseplate:2
- Mate:243: PBG52522-Step:1 ↔ XRN-B1_M-Micrometer-Baseplate:2
- [Mate]: XRN25P_M:2 ↔ XRN-B1_M-Micrometer-Baseplate:1
- [Mate]: XRN25P_M:2 ↔ XRN-B1_M-Micrometer-Baseplate:1
- [Mate]: XRN25P_M:2
- Mate:250
- Mate:251
- Mate:254: KCB1E_M:4
- Mate:255: KCB1E_M:4
- Mate:256: KCB1E_M:5
- Mate:258: KCB1E_M:4 ↔ BBE1-E02-Step:5
- Mate:259: KCB1E_M:4 ↔ BBE1-E02-Step:5
- Mate:261: KCB1E_M:5 ↔ BBE1-E02-Step:4
- Mate:262
- Mate:263
- Mate:272: TR75M:2 ↔ PH75_M-Step:2
- Mate:278: TR75M:4 ↔ PH75_M-Step:3
- Mate:344: 60mm-blank-cageplate-LCP03M-Nikon-MOD:1 ↔ F-Mount-AdapterSM2NFM-Step:1
- Mate:345: 60mm-blank-cageplate-LCP03M-Nikon-MOD:1 ↔ F-Mount-AdapterSM2NFM-Step:1
- Mate:346: F-Mount-AdapterSM2NFM-Step:1 ↔ 50mm_1_4G_body_disassembled:1
- Mate:347: 60mm-blank-cageplate-LCP03M-Nikon-MOD:1 ↔ 50mm_1_4G_body_disassembled:1
- Flush:66: 60mm-blank-cageplate-LCP03M-Nikon-MOD:1 ↔ ER4_CageRod:12
- Mate:350: 60mm-blank-cageplate-LCP03M-Nikon-MOD:1 ↔ ER4_CageRod:13
- Flush:67: 60mm-blank-cageplate-LCP03M-Nikon-MOD:1 ↔ ER4_CageRod:13
- Mate:358: 60mm-blank-cageplate-LCP03M-Nikon-MOD:2 ↔ F-Mount-AdapterSM2NFM-Step:2
- Mate:359: 60mm-blank-cageplate-LCP03M-Nikon-MOD:2 ↔ F-Mount-AdapterSM2NFM-Step:2
- Mate:360: F-Mount-AdapterSM2NFM-Step:2 ↔ 50mm_1_4G_body_disassembled:2
- Mate:361: 60mm-blank-cageplate-LCP03M-Nikon-MOD:2 ↔ 50mm_1_4G_body_disassembled:2
- Mate:365: 60mm-blank-cageplate-LCP03M-Nikon-MOD:2 ↔ ER4_CageRod:14
- Flush:70: 60mm-blank-cageplate-LCP03M-Nikon-MOD:2 ↔ ER4_CageRod:14
- Flush:71: 60mm-blank-cageplate-LCP03M-Nikon-MOD:2 ↔ ER4_CageRod:16
- Mate:366: 60mm-blank-cageplate-LCP03M-Nikon-MOD:2 ↔ ER4_CageRod:16
- Mate:367: TR40M:5 ↔ C60-3060-CMR - 3060 C-MOUNT ROTATING ASSEMBLY_C60-3060-CMR-Mo-ER20:1
- VerticalPos [Mate] (6 mm): TR40M:5 ↔ C60-3060-CMR - 3060 C-MOUNT ROTATING ASSEMBLY_C60-3060-CMR-Mo-ER20:1
- [Mate]: TR40M:5 ↔ KB25_M-Step:1
- [Mate]: TR40M:5 ↔ KB25_M-Step:1
- Angle:44 (0 deg): PBG52522-Step:1 ↔ Cuvette-Sampleholder-with-base:1
- Insert:1 (-6 mm): 60mm-blank-cageplate-LCP03M-Nikon-MOD:1 ↔ ER4_CageRod:19
- Mate:385: PBG52522-Step:1 ↔ ImmersionCuvetteAssembly:1
- Insert:9 (-5 mm): TR40M:5 ↔ Clamp-assembly:1
- Angle:47 (0 deg): PBG52522-Step:1 ↔ Clamp-assembly:1
- Insert:12: SM1A10:1 ↔ EL-16-40-TC-C (133-193-03-R0-01):1
- Insert:13: SM1A10:2 ↔ EL-16-40-TC-C (133-193-03-R0-01):2
- Insert:14: SM1A10:1 ↔ AC254-060-A-ML:1
- Insert:15: SM1M20:1 ↔ AC254-060-A-ML:1
- Insert:16: AC254-060-A-ML_CPY:1 ↔ SM1M20:2
- Insert:17: SM1M20:1 ↔ SM1FCA-APC-Fiberadapter:1
- Insert:18: SM1FCA-APC-Fiberadapter_CPY:1 ↔ SM1M20:2
- Insert:19: PBG52522-Step:1 ↔ RLA150_M:1
- Angle:48 (0 deg): PBG52522-Step:1 ↔ RLA150_M:1
- Mate:386: RLA150_M:1 ↔ FilterWheel-Dynamixel(MX28):1
- Mate:387 (-5 mm): RLA150_M:1 ↔ FilterWheel-Dynamixel(MX28):1
- Mate:388: mirror-bracket:2 ↔ KCB1E_M:5
- Angle:49 (0 deg): PBG52522-Step:1 ↔ mirror-bracket:2
- Mate:389: mirror-bracket:1 ↔ KCB1E_M:4
- Angle:50 (0 deg): PBG52522-Step:1 ↔ mirror-bracket:1
- Insert:20 (-12 mm): 15mm-QS15-galvo-assembly:2 ↔ ER4_CageRod:16
- Insert:21 (-12 mm): 15mm-QS15-galvo-assembly:1 ↔ ER4_CageRod:13
- Flush:74 (45 mm): PBG52522-Step:1 ↔ LS100_Vertical_Assembly:1
- Flush:75 (45 mm): PBG52522-Step:1 ↔ LS100_Vertical_Assembly:2
- Insert:22: CP33_M:13 ↔ AC254-100-A-ML:2
- Insert:23 (-20 mm): CP33_M:13 ↔ ER8_CageRod:5
- Angle:51 (0 deg): CP33_M:5 ↔ CP33_M:13
- Insert:24: Mitutoyo-BD-Plan-Apo-system:1 ↔ Iris15_Volume_Correct:1
- Mate:390: Iris15-XT66P2M:1 ↔ XT66P2_M_single:1
- Flush:76: Iris15-XT66P2M:1 ↔ XT66P2_M_single:1
- Flush:77: Iris15-XT66P2M:1 ↔ XT66P2_M_single:1
- Mate:391: LS100_Vertical_Assembly:1 ↔ AB90H:2
- Mate:392: PBG52522-Step:1 ↔ AB90H:2
- Mate:393: LS100_Vertical_Assembly:1 ↔ AB90H:2
- Mate:394: LS100_Vertical_Assembly:1 ↔ AB90H:1
- Mate:395: PBG52522-Step:1 ↔ AB90H:1
- Flush:78: LS100_Vertical_Assembly:1 ↔ AB90H:1
- Mate:396: LS100_Vertical_Assembly:2 ↔ AB90H:3
- Flush:79: LS100_Vertical_Assembly:2 ↔ AB90H:3
- Mate:397: PBG52522-Step:1 ↔ AB90H:3
- Mate:398: PBG52522-Step:1 ↔ AB90H:4
- Mate:399: LS100_Vertical_Assembly:2 ↔ AB90H:4
- Flush:80: LS100_Vertical_Assembly:2 ↔ AB90H:4
- Mate:400: ThorlabsSM2L30-XT66P2M:1 ↔ XT66P2_M_single:2
- Flush:81: ThorlabsSM2L30-XT66P2M:1 ↔ XT66P2_M_single:2
- Flush:82: ThorlabsSM2L30-XT66P2M:1 ↔ XT66P2_M_single:2
- [Mate]: KB25_M-Step:1 ↔ Cuvette-Sampleholder-with-base:1
- [Mate]: KB25_M-Step:1 ↔ Cuvette-Sampleholder-with-base:1
- [Angle] (0 deg): KB25_M-Step:1 ↔ Cuvette-Sampleholder-with-base:1
- Mate:403: XLN25P_M:1 ↔ XRN-B1_M-Micrometer-Baseplate:2
- Insert:25: Lensagon-T25M-12-155I:1 ↔ Iris15_Volume_Correct:1
- Flush:83: Filter:1 ↔ FilterWheel-Dynamixel(MX28):1
- Insert:26: Filter:3 ↔ FilterWheel-Dynamixel(MX28):1
- Insert:27: Filter:2 ↔ FilterWheel-Dynamixel(MX28):1
